# Autodesk Inventor assembly: Flywheel
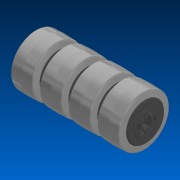
[picture p0: Inventor's stored thumbnail of the model, 180x180]
Saved by Autodesk Inventor 2022.2 (Build 262287000, 287)
## iProperties
Created: 2022-01-05
Part Number: Flywheel
Document SubType Name: Assembly
Designer: omard
Author: omard
## Documents named in this file (2)
- D:\omard\OneDrive - Auburn University\BasketBall Shooting Robot\Flywheel.iam
- D:\omard\OneDrive - Auburn University\BasketBall Shooting Robot\VEX Parts\Colson Performa 3 x 1.5, 1_2 Hex bore (217-4050).ipt
## Components (4 placed, 1 different names)
1. Colson Performa 3 x 1.5, 1_2 Hex bore (217-4050):1 — Flush:1, Flush:4, Mate:2, Mate:3
2. Colson Performa 3 x 1.5, 1_2 Hex bore (217-4050):2 — Flush:2, Flush:5, Mate:1, Mate:2
3. Colson Performa 3 x 1.5, 1_2 Hex bore (217-4050):3 — Flush:3, Flush:6, Mate:3, Angle:1
4. Colson Performa 3 x 1.5, 1_2 Hex bore (217-4050):4 — Flush:1, Flush:2, Flush:3, Flush:4, Flush:5, Flush:6, Mate:1, Angle:1
## Relationships (10: Flush 6, Mate 3, Angle 1)
- Flush:1: Colson Performa 3 x 1.5, 1_2 Hex bore (217-4050):1 ↔ Colson Performa 3 x 1.5, 1_2 Hex bore (217-4050):4
- Flush:2: Colson Performa 3 x 1.5, 1_2 Hex bore (217-4050):2 ↔ Colson Performa 3 x 1.5, 1_2 Hex bore (217-4050):4
- Flush:3: Colson Performa 3 x 1.5, 1_2 Hex bore (217-4050):3 ↔ Colson Performa 3 x 1.5, 1_2 Hex bore (217-4050):4
- Flush:4: Colson Performa 3 x 1.5, 1_2 Hex bore (217-4050):1 ↔ Colson Performa 3 x 1.5, 1_2 Hex bore (217-4050):4
- Flush:5: Colson Performa 3 x 1.5, 1_2 Hex bore (217-4050):2 ↔ Colson Performa 3 x 1.5, 1_2 Hex bore (217-4050):4
- Flush:6: Colson Performa 3 x 1.5, 1_2 Hex bore (217-4050):3 ↔ Colson Performa 3 x 1.5, 1_2 Hex bore (217-4050):4
- Mate:1: Colson Performa 3 x 1.5, 1_2 Hex bore (217-4050):2 ↔ Colson Performa 3 x 1.5, 1_2 Hex bore (217-4050):4
- Mate:2: Colson Performa 3 x 1.5, 1_2 Hex bore (217-4050):1 ↔ Colson Performa 3 x 1.5, 1_2 Hex bore (217-4050):2
- Mate:3: Colson Performa 3 x 1.5, 1_2 Hex bore (217-4050):1 ↔ Colson Performa 3 x 1.5, 1_2 Hex bore (217-4050):3
- Angle:1 (0 deg): Colson Performa 3 x 1.5, 1_2 Hex bore (217-4050):3 ↔ Colson Performa 3 x 1.5, 1_2 Hex bore (217-4050):4
